# Autodesk Inventor assembly: servoconbrazo
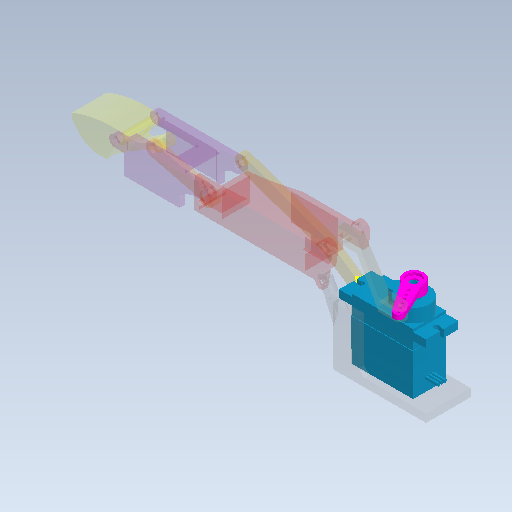
[picture p0: Inventor's stored thumbnail of the model, 512x512]
Saved by Autodesk Inventor 2020 (Build 240168000, 168)
## iProperties
Created: 2021-07-21
Part Number: servoconbrazo
Document SubType Name: Assembly
Designer: chalo
Author: chalo
## Documents named in this file (11)
- C:\Users\chalo\OneDrive\Documents\GitHub\Interfaces-Biomedicas-2021\Gonzalo Palarea\Inventor\servoconbrazo.iam
- C:\Users\chalo\OneDrive\Documents\GitHub\Interfaces-Biomedicas-2021\Gonzalo Palarea\Inventor\referencias\Arm01.ipt
- C:\Users\chalo\OneDrive\Documents\GitHub\Interfaces-Biomedicas-2021\Gonzalo Palarea\Inventor\Base_dedo.ipt
- C:\Users\chalo\OneDrive\Documents\GitHub\Interfaces-Biomedicas-2021\Gonzalo Palarea\Inventor\Union_dedo_base.ipt
- C:\Users\chalo\OneDrive\Documents\GitHub\Interfaces-Biomedicas-2021\Gonzalo Palarea\Inventor\Dedo_1.ipt
- C:\Users\chalo\OneDrive\Documents\GitHub\Interfaces-Biomedicas-2021\Gonzalo Palarea\Inventor\Dedo_2.ipt
- C:\Users\chalo\OneDrive\Documents\GitHub\Interfaces-Biomedicas-2021\Gonzalo Palarea\Inventor\Dedo_3.ipt
- C:\Users\chalo\OneDrive\Documents\GitHub\Interfaces-Biomedicas-2021\Gonzalo Palarea\Inventor\Dedo_4.ipt
- C:\Users\chalo\OneDrive\Documents\GitHub\Interfaces-Biomedicas-2021\Gonzalo Palarea\Inventor\stls\union_yema.ipt
- C:\Users\chalo\OneDrive\Documents\GitHub\Interfaces-Biomedicas-2021\Gonzalo Palarea\Inventor\MG90_Rebuild copy.ipt
- C:\Users\chalo\OneDrive\Documents\GitHub\Interfaces-Biomedicas-2021\Gonzalo Palarea\Inventor\assmtest.iam
## Components (10 placed, 10 different names)
1. MG90_Rebuild copy:1 — Angle:1, Mate:1, Insert:1, Flush:2
2. Arm01:1 — Angle:1, Mate:1, Insert:1, Flush:5, Flush:6
3. Base_dedo:1 — Flush:1, Flush:2, Flush:9, Flush:11
4. Union_dedo_base:1 — Flush:5, Flush:6, Flush:8
5. Dedo_1:1 — Flush:7, Flush:8, Flush:9, Flush:10
6. Dedo_2:1 — Flush:10, Flush:12
7. Dedo_3:1 — Flush:11
8. Dedo_4:1 — Flush:12, Flush:13, Flush:14, Flush:15
9. union_yema:1 — Flush:15
10. assmtest:1 [sub-assembly]
## Relationships (16: Flush 13, Angle 1, Mate 1, Insert 1)
- Angle:1 (30 deg): MG90_Rebuild copy:1 ↔ Arm01:1
- Mate:1: MG90_Rebuild copy:1 ↔ Arm01:1
- Insert:1: MG90_Rebuild copy:1 ↔ Arm01:1
- Flush:1: Base_dedo:1
- Flush:2: MG90_Rebuild copy:1 ↔ Base_dedo:1
- Flush:5: Arm01:1 ↔ Union_dedo_base:1
- Flush:6: Arm01:1 ↔ Union_dedo_base:1
- Flush:7: Dedo_1:1
- Flush:8: Union_dedo_base:1 ↔ Dedo_1:1
- Flush:9: Base_dedo:1 ↔ Dedo_1:1
- Flush:10: Dedo_1:1 ↔ Dedo_2:1
- Flush:11: Base_dedo:1 ↔ Dedo_3:1
- Flush:12: Dedo_2:1 ↔ Dedo_4:1
- Flush:13 (-6.5 mm): Dedo_4:1
- Flush:14: Dedo_4:1
- Flush:15: Dedo_4:1 ↔ union_yema:1
